# Autodesk Inventor assembly: Audio_module
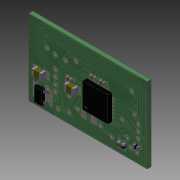
[picture p0: Inventor's stored thumbnail of the model, 180x180]
Saved by Autodesk Inventor 2013 (Build 170138000, 138)
## iProperties
Created: 2015-07-03
Part Number: Audio_module
Document SubType Name: Assembly
Designer: terg
Author: terg
## Documents named in this file (8)
- C:\Users\terg\Projects\ModularElectronics\3D_models\Audio_module\Audio_module.iam
- C:\Users\terg\Projects\ModularElectronics\3D_models\Audio_module\Audio_module_PCB.ipt
- C:\Users\terg\Projects\ModularElectronics\3D_models\Components\0402_cap.ipt
- C:\Users\terg\Projects\ModularElectronics\3D_models\Components\0402_res.ipt
- C:\Users\terg\Projects\ModularElectronics\3D_models\Components\0805_cap.ipt
- C:\Users\terg\Projects\ModularElectronics\3D_models\Components\EFM32ZG110.ipt
- C:\Users\terg\Projects\ModularElectronics\3D_models\Audio_module\ADAU1761.ipt
- C:\Users\terg\Projects\ModularElectronics\3D_models\Audio_module\LTC6905.ipt
## Components (26 placed, 7 different names)
1. Audio_module_PCB:1 — Zestawiający:1, Zestawiający:2, Zestawiający:3, Zestawiający:4, Zestawiający:5, Zestawiający:6, Zestawiający:7, Równoległy:1, Równoległy:2, Równoległy:3, Równoległy:4, Równoległy:5, Równoległy:6, Równoległy:7, Równoległy:8, Równoległy:9, Równoległy:10, Równoległy:11, Równoległy:12, Równoległy:13, Równoległy:14, Zestawiający:8, Zestawiający:9, Zestawiający:10, Zestawiający:11, Zestawiający:12, Zestawiający:13, Równoległy:15, Równoległy:16, Równoległy:17, Równoległy:18, Równoległy:19, Równoległy:20, Równoległy:21, Równoległy:22, Równoległy:23, Równoległy:24, Równoległy:25, Równoległy:26, Zestawiający:14, Zestawiający:15, Zestawiający:16, Zestawiający:17, Zestawiający:18, Zestawiający:19, Zestawiający:20, Zestawiający:21, Zestawiający:22, Równoległy:27, Równoległy:28, Równoległy:29, Równoległy:30, Równoległy:31, Równoległy:32, Równoległy:33, Równoległy:34, Równoległy:35, Równoległy:36, Równoległy:37, Równoległy:38, Równoległy:39, Równoległy:40, Równoległy:41, Równoległy:42, Równoległy:43, Równoległy:44, Zestawiający:23, Równoległy:45, Równoległy:46, Zestawiający:24, Równoległy:47, Równoległy:48, Zestawiający:25, Równoległy:49, Równoległy:50
2. 0402_cap:1 — Zestawiający:2, Równoległy:1, Równoległy:2
3. 0402_cap:2 — Zestawiający:1, Równoległy:3, Równoległy:14
4. 0402_cap:3 — Zestawiający:3, Równoległy:5, Równoległy:7
5. 0402_cap:4 — Zestawiający:4, Równoległy:4, Równoległy:6
6. 0402_cap:5 — Zestawiający:5, Równoległy:8, Równoległy:13
7. 0402_cap:6 — Zestawiający:6, Równoległy:9, Równoległy:12
8. 0402_res:1 — Zestawiający:7, Równoległy:10, Równoległy:11
9. 0805_cap:1 — Zestawiający:8, Równoległy:15, Równoległy:16
10. 0805_cap:2 — Zestawiający:10, Równoległy:19, Równoległy:22
11. 0805_cap:3 — Zestawiający:11, Równoległy:17, Równoległy:25
12. 0805_cap:4 — Zestawiający:13, Równoległy:23, Równoległy:24
13. 0805_cap:5 — Zestawiający:12, Równoległy:20, Równoległy:21
14. 0805_cap:6 — Zestawiający:9, Równoległy:18, Równoległy:26
15. 0402_res:2 — Zestawiający:14, Równoległy:29, Równoległy:32
16. 0402_cap:7 — Zestawiający:18, Równoległy:38, Równoległy:40
17. 0402_cap:8 — Zestawiający:19, Równoległy:37, Równoległy:39
18. 0402_cap:9 — Zestawiający:17, Równoległy:42, Równoległy:43
19. 0402_cap:10 — Zestawiający:16, Równoległy:35, Równoległy:36
20. 0402_res:3 — Zestawiający:15, Równoległy:27, Równoległy:28
21. 0402_cap:11 — Zestawiający:20, Równoległy:30, Równoległy:31
22. 0805_cap:7 — Zestawiający:21, Równoległy:41, Równoległy:44
23. 0805_cap:8 — Zestawiający:22, Równoległy:33, Równoległy:34
24. EFM32ZG110:1 — Zestawiający:23, Równoległy:45, Równoległy:46
25. ADAU1761:1 — Zestawiający:24, Równoległy:47, Równoległy:48
26. LTC6905:1 — Zestawiający:25, Równoległy:49, Równoległy:50
## Relationships (75: Flush 50, Mate 25)
- Zestawiający:1 [Mate]: Audio_module_PCB:1 ↔ 0402_cap:2
- Zestawiający:2 [Mate]: Audio_module_PCB:1 ↔ 0402_cap:1
- Zestawiający:3 [Mate]: Audio_module_PCB:1 ↔ 0402_cap:3
- Zestawiający:4 [Mate]: Audio_module_PCB:1 ↔ 0402_cap:4
- Zestawiający:5 [Mate]: Audio_module_PCB:1 ↔ 0402_cap:5
- Zestawiający:6 [Mate]: Audio_module_PCB:1 ↔ 0402_cap:6
- Zestawiający:7 [Mate]: Audio_module_PCB:1 ↔ 0402_res:1
- Równoległy:1 [Flush] (3.831 mm): Audio_module_PCB:1 ↔ 0402_cap:1
- Równoległy:2 [Flush] (4.553 mm): Audio_module_PCB:1 ↔ 0402_cap:1
- Równoległy:3 [Flush] (5.675 mm): Audio_module_PCB:1 ↔ 0402_cap:2
- Równoległy:4 [Flush] (11.679 mm): Audio_module_PCB:1 ↔ 0402_cap:4
- Równoległy:5 [Flush] (11.688 mm): Audio_module_PCB:1 ↔ 0402_cap:3
- Równoległy:6 [Flush] (3.019 mm): Audio_module_PCB:1 ↔ 0402_cap:4
- Równoległy:7 [Flush] (4.006 mm): Audio_module_PCB:1 ↔ 0402_cap:3
- Równoległy:8 [Flush] (9.3 mm): Audio_module_PCB:1 ↔ 0402_cap:5
- Równoległy:9 [Flush] (9.274 mm): Audio_module_PCB:1 ↔ 0402_cap:6
- Równoległy:10 [Flush] (9.253 mm): Audio_module_PCB:1 ↔ 0402_res:1
- Równoległy:11 [Flush] (-5.713 mm): Audio_module_PCB:1 ↔ 0402_res:1
- Równoległy:12 [Flush] (7.036 mm): Audio_module_PCB:1 ↔ 0402_cap:6
- Równoległy:13 [Flush] (7.945 mm): Audio_module_PCB:1 ↔ 0402_cap:5
- Równoległy:14 [Flush] (3.793 mm): Audio_module_PCB:1 ↔ 0402_cap:2
- Zestawiający:8 [Mate]: Audio_module_PCB:1 ↔ 0805_cap:1
- Zestawiający:9 [Mate]: Audio_module_PCB:1 ↔ 0805_cap:6
- Zestawiający:10 [Mate]: Audio_module_PCB:1 ↔ 0805_cap:2
- Zestawiający:11 [Mate]: Audio_module_PCB:1 ↔ 0805_cap:3
- Zestawiający:12 [Mate]: Audio_module_PCB:1 ↔ 0805_cap:5
- Zestawiający:13 [Mate]: Audio_module_PCB:1 ↔ 0805_cap:4
- Równoległy:15 [Flush] (3.58 mm): Audio_module_PCB:1 ↔ 0805_cap:1
- Równoległy:16 [Flush] (10.857 mm): Audio_module_PCB:1 ↔ 0805_cap:1
- Równoległy:17 [Flush] (2.062 mm): Audio_module_PCB:1 ↔ 0805_cap:3
- Równoległy:18 [Flush] (2.02 mm): Audio_module_PCB:1 ↔ 0805_cap:6
- Równoległy:19 [Flush] (3.489 mm): Audio_module_PCB:1 ↔ 0805_cap:2
- Równoległy:20 [Flush] (17.018 mm): Audio_module_PCB:1 ↔ 0805_cap:5
- Równoległy:21 [Flush] (1.951 mm): Audio_module_PCB:1 ↔ 0805_cap:5
- Równoległy:22 [Flush] (13.469 mm): Audio_module_PCB:1 ↔ 0805_cap:2
- Równoległy:23 [Flush] (13.081 mm): Audio_module_PCB:1 ↔ 0805_cap:4
- Równoległy:24 [Flush] (1.212 mm): Audio_module_PCB:1 ↔ 0805_cap:4
- Równoległy:25 [Flush] (7.951 mm): Audio_module_PCB:1 ↔ 0805_cap:3
- Równoległy:26 [Flush] (9.709 mm): Audio_module_PCB:1 ↔ 0805_cap:6
- Zestawiający:14 [Mate]: Audio_module_PCB:1 ↔ 0402_res:2
- Zestawiający:15 [Mate]: Audio_module_PCB:1 ↔ 0402_res:3
- Zestawiający:16 [Mate]: Audio_module_PCB:1 ↔ 0402_cap:10
- Zestawiający:17 [Mate]: Audio_module_PCB:1 ↔ 0402_cap:9
- Zestawiający:18 [Mate]: Audio_module_PCB:1 ↔ 0402_cap:7
- Zestawiający:19 [Mate]: Audio_module_PCB:1 ↔ 0402_cap:8
- Zestawiający:20 [Mate]: Audio_module_PCB:1 ↔ 0402_cap:11
- Zestawiający:21 [Mate]: Audio_module_PCB:1 ↔ 0805_cap:7
- Zestawiający:22 [Mate]: Audio_module_PCB:1 ↔ 0805_cap:8
- Równoległy:27 [Flush] (1.378 mm): Audio_module_PCB:1 ↔ 0402_res:3
- Równoległy:28 [Flush] (2.739 mm): Audio_module_PCB:1 ↔ 0402_res:3
- Równoległy:29 [Flush] (1.225 mm): Audio_module_PCB:1 ↔ 0402_res:2
- Równoległy:30 [Flush] (1.186 mm): Audio_module_PCB:1 ↔ 0402_cap:11
- Równoległy:31 [Flush] (5.12 mm): Audio_module_PCB:1 ↔ 0402_cap:11
- Równoległy:32 [Flush] (4.222 mm): Audio_module_PCB:1 ↔ 0402_res:2
- Równoległy:33 [Flush] (13.623 mm): Audio_module_PCB:1 ↔ 0805_cap:8
- Równoległy:34 [Flush] (6.078 mm): Audio_module_PCB:1 ↔ 0805_cap:8
- Równoległy:35 [Flush] (14.718 mm): Audio_module_PCB:1 ↔ 0402_cap:10
- Równoległy:36 [Flush] (7.765 mm): Audio_module_PCB:1 ↔ 0402_cap:10
- Równoległy:37 [Flush] (8.158 mm): Audio_module_PCB:1 ↔ 0402_cap:8
- Równoległy:38 [Flush] (10.037 mm): Audio_module_PCB:1 ↔ 0402_cap:7
- Równoległy:39 [Flush] (10.391 mm): Audio_module_PCB:1 ↔ 0402_cap:8
- Równoległy:40 [Flush] (10.366 mm): Audio_module_PCB:1 ↔ 0402_cap:7
- Równoległy:41 [Flush] (20.034 mm): Audio_module_PCB:1 ↔ 0805_cap:7
- Równoległy:42 [Flush] (21.054 mm): Audio_module_PCB:1 ↔ 0402_cap:9
- Równoległy:43 [Flush] (4.558 mm): Audio_module_PCB:1 ↔ 0402_cap:9
- Równoległy:44 [Flush] (5.497 mm): Audio_module_PCB:1 ↔ 0805_cap:7
- Zestawiający:23 [Mate]: Audio_module_PCB:1 ↔ EFM32ZG110:1
- Równoległy:45 [Flush] (4.632 mm): Audio_module_PCB:1 ↔ EFM32ZG110:1
- Równoległy:46 [Flush] (6.965 mm): Audio_module_PCB:1 ↔ EFM32ZG110:1
- Zestawiający:24 [Mate]: Audio_module_PCB:1 ↔ ADAU1761:1
- Równoległy:47 [Flush] (4.622 mm): Audio_module_PCB:1 ↔ ADAU1761:1
- Równoległy:48 [Flush] (6.894 mm): Audio_module_PCB:1 ↔ ADAU1761:1
- Zestawiający:25 [Mate]: Audio_module_PCB:1 ↔ LTC6905:1
- Równoległy:49 [Flush] (1.232 mm): Audio_module_PCB:1 ↔ LTC6905:1
- Równoległy:50 [Flush] (1.459 mm): Audio_module_PCB:1 ↔ LTC6905:1
